# Autodesk Inventor assembly: Assemblyframe buiten
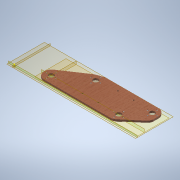
[picture p0: Inventor's stored thumbnail of the model, 180x180]
Saved by Autodesk Inventor 2021 (Build 250183000, 183)
## iProperties
Manager: PJ / DCS
Company: Emmaüs Bovenbouw Aalter
Created: 2021-03-07
Part Number: Assemblyframe buiten
Catalog Web Link: http://emmausbovenbouw.op-weg.be/
Vendor: Emmaüs Bovenbouw Aalter
Document SubType Name: Assembly
Designer: Antho
Engineer: Declercq St.
Authority: Declercq St.
Title: Algemene Projecttitel
Author: Antho
## Documents named in this file (3)
- C:\Users\Antho\OneDrive\Documenten\Inventor\Inventor\GIP 6EM\Assembly\A1\Assemblyframe buiten.iam
- C:\Users\Antho\OneDrive\Documenten\Inventor\Inventor\GIP 6EM\Wielen\Frame wiel.ipt
- C:\Users\Antho\OneDrive\Documenten\Inventor\Inventor\GIP 6EM\Wielen\Kogel houders.ipt
## Components (2 placed, 2 different names)
1. Frame wiel:1 — Mate:1, Mate:2, Flush:1
2. Kogel houders:1 — Mate:1, Mate:2, Flush:1
## Relationships (3: Mate 2, Flush 1)
- Mate:1: Frame wiel:1 ↔ Kogel houders:1
- Mate:2: Frame wiel:1 ↔ Kogel houders:1
- Flush:1: Frame wiel:1 ↔ Kogel houders:1
